# Autodesk Inventor assembly: Head
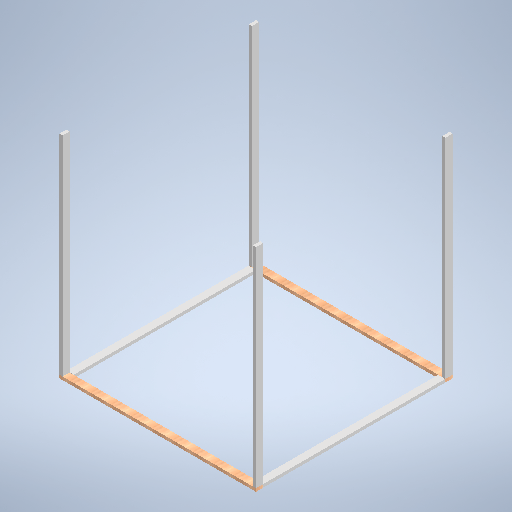
[picture p0: Inventor's stored thumbnail of the model, 512x512]
Saved by Autodesk Inventor 2025 (Build 290162000, 162)
## iProperties
Created: 2024-09-18
Part Number: Head
Document SubType Name: Assembly
Designer: localadmin
Author: localadmin
## Documents named in this file (4)
- C:\Users\localadmin\Documents\USCTigerBurn24\Head.iam
- C:\Users\localadmin\Documents\USCTigerBurn24\Standard Timber\2x4x96.ipt
- C:\Users\localadmin\Documents\USCTigerBurn24\Standard Timber\7'5''x2x4Correct.ipt
- C:\Users\localadmin\Documents\USCTigerBurn24\Standard Timber\10'x2x4.ipt
## Components (8 placed, 3 different names)
1. 2x4x96:1 — Flush:1, Mate:1, Flush:2, Mate:2, Flush:3, Flush:4, Mate:3, Flush:7, Flush:8, Mate:5, Flush:11, Flush:12, Mate:7, Flush:15, Flush:16
2. 2x4x96:2 — Flush:1, Mate:1, Flush:2, Flush:5, Flush:6, Mate:4, Flush:9, Flush:10, Mate:6, Flush:13, Flush:14
3. 7'5''x2x4Correct:1 — Mate:2, Flush:3, Flush:4, Flush:5, Flush:6
4. 7'5''x2x4Correct:2 — Mate:3, Flush:7, Flush:8
5. 10'x2x4:1 — Mate:4, Flush:9, Flush:10
6. 10'x2x4:2 — Mate:5, Flush:11, Flush:12
7. 10'x2x4:3 — Mate:6, Flush:13, Flush:14
8. 10'x2x4:4 — Mate:7, Flush:15, Flush:16
## Relationships (23: Flush 16, Mate 7)
- Flush:1: 2x4x96:1 ↔ 2x4x96:2
- Mate:1 (2260.6 mm): 2x4x96:1 ↔ 2x4x96:2
- Flush:2: 2x4x96:1 ↔ 2x4x96:2
- Mate:2: 2x4x96:1 ↔ 7'5''x2x4Correct:1
- Flush:3: 2x4x96:1 ↔ 7'5''x2x4Correct:1
- Flush:4: 2x4x96:1 ↔ 7'5''x2x4Correct:1
- Flush:5: 2x4x96:2 ↔ 7'5''x2x4Correct:1
- Flush:6: 2x4x96:2 ↔ 7'5''x2x4Correct:1
- Mate:3: 2x4x96:1 ↔ 7'5''x2x4Correct:2
- Flush:7: 2x4x96:1 ↔ 7'5''x2x4Correct:2
- Flush:8: 2x4x96:1 ↔ 7'5''x2x4Correct:2
- Mate:4: 2x4x96:2 ↔ 10'x2x4:1
- Flush:9: 2x4x96:2 ↔ 10'x2x4:1
- Flush:10: 2x4x96:2 ↔ 10'x2x4:1
- Mate:5: 2x4x96:1 ↔ 10'x2x4:2
- Flush:11: 2x4x96:1 ↔ 10'x2x4:2
- Flush:12: 2x4x96:1 ↔ 10'x2x4:2
- Mate:6: 2x4x96:2 ↔ 10'x2x4:3
- Flush:13: 2x4x96:2 ↔ 10'x2x4:3
- Flush:14: 2x4x96:2 ↔ 10'x2x4:3
- Mate:7: 2x4x96:1 ↔ 10'x2x4:4
- Flush:15: 2x4x96:1 ↔ 10'x2x4:4
- Flush:16: 2x4x96:1 ↔ 10'x2x4:4
